# Autodesk Inventor assembly: Servo 60KG
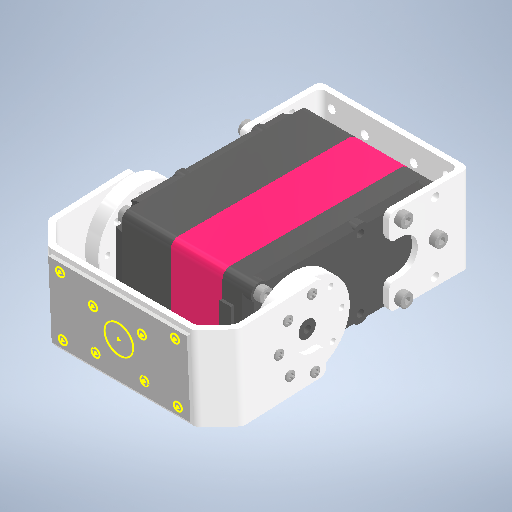
[picture p0: Inventor's stored thumbnail of the model, 512x512]
Saved by Autodesk Inventor 2025.1 (Build 291241000, 241)
## iProperties
Created: 2024-12-01
Part Number: Servo 60KG
Document SubType Name: Assembly
Designer: Cristhian Vigo
Author: Cristhian Vigo
## Documents named in this file (14)
- D:\CRISTHIAN\universidad\ciclo 8\Robótica\PROYECTO\Modelo\ROBOT_5GDL\Servo 60KG.iam
- D:\CRISTHIAN\universidad\ciclo 8\Robótica\PROYECTO\Modelo\ROBOT_5GDL\base.ipt
- D:\CRISTHIAN\universidad\ciclo 8\Robótica\PROYECTO\Modelo\ROBOT_5GDL\Servo.ipt
- D:\CRISTHIAN\universidad\ciclo 8\Robótica\PROYECTO\Modelo\ROBOT_5GDL\base giratoria.ipt
- D:\CRISTHIAN\universidad\ciclo 8\Robótica\PROYECTO\Modelo\ROBOT_5GDL\DIN_EN_ISO_4762_M2,5x5.ipt v2.ipt
- D:\CRISTHIAN\universidad\ciclo 8\Robótica\PROYECTO\Modelo\ROBOT_5GDL\DIN_EN_ISO_4762_M2,5x25.ipt v2.ipt
- D:\CRISTHIAN\universidad\ciclo 8\Robótica\PROYECTO\Modelo\ROBOT_5GDL\engranaje recto servo.ipt
- D:\CRISTHIAN\universidad\ciclo 8\Robótica\PROYECTO\Modelo\ROBOT_5GDL\rodamiento.ipt
- D:\CRISTHIAN\universidad\ciclo 8\Robótica\PROYECTO\Modelo\ROBOT_5GDL\Screw 3 v1.ipt
- D:\CRISTHIAN\universidad\ciclo 8\Robótica\PROYECTO\Modelo\ROBOT_5GDL\Soporte 1.ipt
- D:\CRISTHIAN\universidad\ciclo 8\Robótica\PROYECTO\Modelo\ROBOT_5GDL\Soporte 2.ipt
- D:\CRISTHIAN\universidad\ciclo 8\Robótica\PROYECTO\Modelo\ROBOT_5GDL\Part2.ipt
- DIN_EN_ISO_4762_M2,5x5.ipt
- DIN_EN_ISO_4762_M2,5x25.ipt
## Components (28 placed, 11 different names)
1. base:1 — Insert:7, Insert:8, Mate:6
2. Servo:1 — Flush:1, Mate:1, Mate:2, Mate:3, Insert:8, Insert:17, Insert:19, Insert:20, Insert:21, Insert:22
3. base giratoria:1 — Insert:18, Mate:4, Mate:5
4. DIN_EN_ISO_4762_M2,5x5.ipt v2:1 — Insert:1
5. DIN_EN_ISO_4762_M2,5x25.ipt v2:1 — Insert:19
6. engranaje recto servo:1 — Insert:17, Insert:18
7. rodamiento:1 — Insert:7
8. Soporte 1:1 — Mate:4, Mate:5, Mate:6, Insert:23, Insert:24, Insert:26, Insert:28, Insert:30, Insert:31, Insert:32, Insert:33, Insert:34, Insert:35, Mate:7
9. Soporte 2:1 — Mate:1, Mate:2, Mate:3, Insert:1, Insert:2, Insert:3, Insert:4, Insert:5, Insert:6
10. DIN_EN_ISO_4762_M2,5x5.ipt v2:2 — Insert:2
11. DIN_EN_ISO_4762_M2,5x5.ipt v2:3 — Insert:3
12. DIN_EN_ISO_4762_M2,5x5.ipt v2:4 — Insert:5
13. DIN_EN_ISO_4762_M2,5x5.ipt v2:5 — Insert:4
14. DIN_EN_ISO_4762_M2,5x5.ipt v2:6 — Insert:6
15. DIN_EN_ISO_4762_M2,5x25.ipt v2:2 — Insert:21
16. DIN_EN_ISO_4762_M2,5x25.ipt v2:3 — Insert:22
17. DIN_EN_ISO_4762_M2,5x25.ipt v2:4 — Insert:20
18. Screw 3 v1:11 — Insert:30
19. Screw 3 v1:12 — Insert:28
20. Screw 3 v1:13 — Insert:26
21. Screw 3 v1:14 — Insert:23
22. Screw 3 v1:15 — Insert:24
23. Screw 3 v1:16 — Insert:32
24. Screw 3 v1:17 — Insert:31
25. Screw 3 v1:18 — Insert:33
26. Screw 3 v1:19 — Insert:35
27. Screw 3 v1:20 — Insert:34
28. Part2:1 — Mate:7
## Relationships (32: Insert 24, Mate 7, Flush 1)
- Flush:1 (-23.8125 mm): Servo:1
- Mate:1: Servo:1 ↔ Soporte 2:1
- Mate:2: Servo:1 ↔ Soporte 2:1
- Mate:3: Servo:1 ↔ Soporte 2:1
- Insert:1: DIN_EN_ISO_4762_M2,5x5.ipt v2:1 ↔ Soporte 2:1
- Insert:2: Soporte 2:1 ↔ DIN_EN_ISO_4762_M2,5x5.ipt v2:2
- Insert:3: Soporte 2:1 ↔ DIN_EN_ISO_4762_M2,5x5.ipt v2:3
- Insert:4: Soporte 2:1 ↔ DIN_EN_ISO_4762_M2,5x5.ipt v2:5
- Insert:5: Soporte 2:1 ↔ DIN_EN_ISO_4762_M2,5x5.ipt v2:4
- Insert:6: Soporte 2:1 ↔ DIN_EN_ISO_4762_M2,5x5.ipt v2:6
- Insert:7: base:1 ↔ rodamiento:1
- Insert:8: base:1 ↔ Servo:1
- Insert:17: Servo:1 ↔ engranaje recto servo:1
- Insert:18: base giratoria:1 ↔ engranaje recto servo:1
- Insert:19: Servo:1 ↔ DIN_EN_ISO_4762_M2,5x25.ipt v2:1
- Insert:20: Servo:1 ↔ DIN_EN_ISO_4762_M2,5x25.ipt v2:4
- Insert:21: Servo:1 ↔ DIN_EN_ISO_4762_M2,5x25.ipt v2:2
- Insert:22: Servo:1 ↔ DIN_EN_ISO_4762_M2,5x25.ipt v2:3
- Mate:4: base giratoria:1 ↔ Soporte 1:1
- Mate:5: base giratoria:1 ↔ Soporte 1:1
- Mate:6: base:1 ↔ Soporte 1:1
- Insert:23: Soporte 1:1 ↔ Screw 3 v1:14
- Insert:24: Soporte 1:1 ↔ Screw 3 v1:15
- Insert:26: Soporte 1:1 ↔ Screw 3 v1:13
- Insert:28: Soporte 1:1 ↔ Screw 3 v1:12
- Insert:30: Soporte 1:1 ↔ Screw 3 v1:11
- Insert:31: Soporte 1:1 ↔ Screw 3 v1:17
- Insert:32: Soporte 1:1 ↔ Screw 3 v1:16
- Insert:33: Soporte 1:1 ↔ Screw 3 v1:18
- Insert:34: Soporte 1:1 ↔ Screw 3 v1:20
- Insert:35: Soporte 1:1 ↔ Screw 3 v1:19
- Mate:7: Soporte 1:1 ↔ Part2:1
